# Autodesk Inventor assembly: new assembly
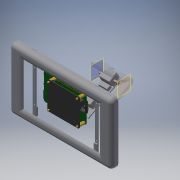
[picture p0: Inventor's stored thumbnail of the model, 180x180]
Saved by Autodesk Inventor 2018 (Build 220112000, 112)
## iProperties
Created: 2019-09-14
Part Number: new assembly
Document SubType Name: Assembly
Designer: Jacob
Author: Jacob
## Documents named in this file (10)
- C:\Users\Jacob\git_repos\POE-AIO\CAD Files\new assembly.iam
- C:\Users\Jacob\git_repos\POE-AIO\CAD Files\Official parts\raspberry pi display.ipt
- C:\Users\Jacob\git_repos\POE-AIO\CAD Files\Better designed front piece.ipt
- C:\Users\Jacob\git_repos\POE-AIO\CAD Files\better support stick.ipt
- C:\Users\Jacob\git_repos\POE-AIO\CAD Files\Official parts\Raspberry Pi 3 .ipt
- C:\Users\Jacob\git_repos\POE-AIO\CAD Files\Official parts\Stand off.ipt
- C:\Users\Jacob\git_repos\POE-AIO\CAD Files\Official parts\raspberry pi display module.ipt
- C:\Users\Jacob\git_repos\POE-AIO\CAD Files\Better designed Triangular Prisim back part.ipt
- C:\Users\Jacob\git_repos\POE-AIO\CAD Files\More powerful POE Splitter.ipt
- C:\Users\Jacob\git_repos\POE-AIO\CAD Files\Ethernet connector.ipt
## Components (13 placed, 9 different names)
1. raspberry pi display:1 — Mate:1, Mate:2, Mate:3, Mate:4, Mate:5, Mate:6, Mate:7, Mate:8, Mate:9, Mate:10, Mate:11, Mate:12
2. Better designed front piece:1 — Mate:1, Mate:2, Mate:3, Mate:29, Flush:1, Mate:30
3. better support stick:1 — Mate:4, Mate:5, Mate:9
4. better support stick:2 — Mate:6, Mate:7, Mate:8
5. Raspberry Pi 3 :1 — Mate:26, Mate:27, Mate:28
6. Stand off:1 — Mate:15, Mate:16, Mate:27
7. Stand off:2 — Mate:13, Mate:14, Mate:26
8. Stand off:3 — Mate:17, Mate:18, Mate:28
9. Stand off:4 — Mate:19, Mate:20
10. raspberry pi display module:1 — Mate:10, Mate:11, Mate:12, Mate:13, Mate:14, Mate:15, Mate:16, Mate:17, Mate:18, Mate:19, Mate:20
11. Better designed Triangular Prisim back part:1 — Mate:29, Flush:1, Mate:30, Mate:31, Mate:32, Mate:33
12. More powerful POE Splitter:1 — Mate:31, Mate:32, Mate:33, Mate:34, Mate:35, Mate:36
13. Ethernet connector:1 — Mate:34, Mate:35, Mate:36
## Relationships (32: Mate 31, Flush 1)
- Mate:1 (1 mm): raspberry pi display:1 ↔ Better designed front piece:1
- Mate:2: raspberry pi display:1 ↔ Better designed front piece:1
- Mate:3 (0.5 mm): raspberry pi display:1 ↔ Better designed front piece:1
- Mate:4: raspberry pi display:1 ↔ better support stick:1
- Mate:5: raspberry pi display:1 ↔ better support stick:1
- Mate:6: raspberry pi display:1 ↔ better support stick:2
- Mate:7: raspberry pi display:1 ↔ better support stick:2
- Mate:8: raspberry pi display:1 ↔ better support stick:2
- Mate:9: raspberry pi display:1 ↔ better support stick:1
- Mate:10: raspberry pi display:1 ↔ raspberry pi display module:1
- Mate:11: raspberry pi display:1 ↔ raspberry pi display module:1
- Mate:12: raspberry pi display:1 ↔ raspberry pi display module:1
- Mate:13: Stand off:2 ↔ raspberry pi display module:1
- Mate:14: Stand off:2 ↔ raspberry pi display module:1
- Mate:15: Stand off:1 ↔ raspberry pi display module:1
- Mate:16: Stand off:1 ↔ raspberry pi display module:1
- Mate:17: Stand off:3 ↔ raspberry pi display module:1
- Mate:18: Stand off:3 ↔ raspberry pi display module:1
- Mate:19: Stand off:4 ↔ raspberry pi display module:1
- Mate:20: Stand off:4 ↔ raspberry pi display module:1
- Mate:26: Raspberry Pi 3 :1 ↔ Stand off:2
- Mate:27: Raspberry Pi 3 :1 ↔ Stand off:1
- Mate:28: Raspberry Pi 3 :1 ↔ Stand off:3
- Mate:29: Better designed front piece:1 ↔ Better designed Triangular Prisim back part:1
- Flush:1: Better designed front piece:1 ↔ Better designed Triangular Prisim back part:1
- Mate:30: Better designed front piece:1 ↔ Better designed Triangular Prisim back part:1
- Mate:31: Better designed Triangular Prisim back part:1 ↔ More powerful POE Splitter:1
- Mate:32: Better designed Triangular Prisim back part:1 ↔ More powerful POE Splitter:1
- Mate:33: Better designed Triangular Prisim back part:1 ↔ More powerful POE Splitter:1
- Mate:34: More powerful POE Splitter:1 ↔ Ethernet connector:1
- Mate:35: More powerful POE Splitter:1 ↔ Ethernet connector:1
- Mate:36: More powerful POE Splitter:1 ↔ Ethernet connector:1
